# Autodesk Inventor assembly: Short-Cage
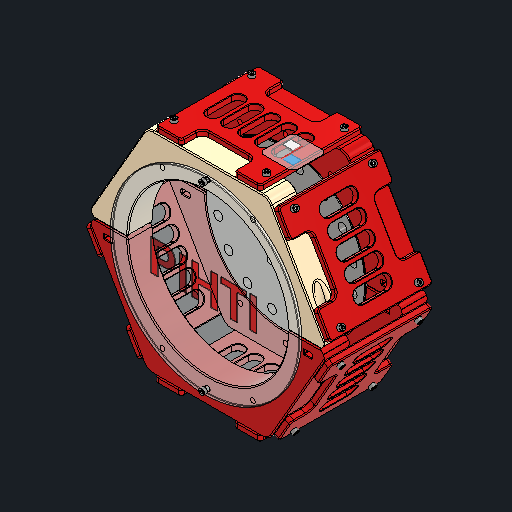
[picture p0: Inventor's stored thumbnail of the model, 512x512]
Saved by Autodesk Inventor 2026 (Build 300175050, 175E)
## iProperties
Created: 2024-07-04
Part Number: Short-Cage
Document SubType Name: Assembly
Designer: kuzmin
Author: kuzmin
## Documents named in this file (8)
- C:\Users\queezz\Dropbox\Drawings\PIHTI\Plasma Vessel\Cathode-Flange-Cage\Short-Cage.iam
- C:\Users\queezz\Dropbox\Drawings\PIHTI\Plasma Vessel\Cathode-Flange-Cage\Baseplate-for-ICF152-flange-outer-part-bottom.ipt
- C:\Users\queezz\Dropbox\Drawings\PIHTI\Plasma Vessel\Cathode-Flange-Cage\Cover-Plate-short-with-bolts.iam
- C:\Users\queezz\Dropbox\Drawings\PIHTI\ContentCenter\CF-parts\CF-Flanges\CF_152-70.ipt
- C:\Users\queezz\Dropbox\Drawings\PIHTI\Plasma Vessel\Cathode-Flange-Cage\cage-disk-lid.ipt
- C:\Users\queezz\Dropbox\Drawings\PIHTI\ContentCenter\Fastners\M3x10-SHCS.ipt
- C:\Users\queezz\Dropbox\Drawings\PIHTI\ContentCenter\Fastners\brass-insert-m3x5.ipt
- C:\Users\queezz\Dropbox\Drawings\PIHTI\Plasma Vessel\Cathode-Flange-Cage\Baseplate-for-ICF152-flange-outer-part-top-v2.ipt
## Components (17 placed, 7 different names)
1. Baseplate-for-ICF152-flange-outer-part-bottom:1 — Rigid:1, Rigid:6, Rigid:7, Rigid:8
2. Baseplate-for-ICF152-flange-outer-part-bottom:2 — Rigid:1, Mate:5, Rigid:3
3. Baseplate-for-ICF152-flange-outer-part-bottom:4 — Mate:5
4. CF_152-70:1 — Rigid:3
5. cage-disk-lid:1 — Rigid:4, Rigid:5, Rigid:9
6. Baseplate-for-ICF152-flange-outer-part-top-v2:1 — Rigid:9
7. JIS B 1176 - Metric M3 x 10:1 — Rigid:5
8. JIS B 1176 - Metric M3 x 10:2 — Rigid:4
9. brass-insert-m3x5:1
10. brass-insert-m3x5:2 — Rigid:6
11. brass-insert-m3x5:3 — Rigid:7
12. brass-insert-m3x5:4
13. Cover-Plate-short-with-bolts:1 [sub-assembly] — Rigid:8
14. Cover-Plate-short-with-bolts:2 [sub-assembly]
15. Cover-Plate-short-with-bolts:3 [sub-assembly]
16. Cover-Plate-short-with-bolts:4 [sub-assembly]
17. Cover-Plate-short-with-bolts:5 [sub-assembly]
## Component patterns: (5 elements, first: Cover-Plate-short-with-bolts:1)
## Relationships (10: WeldJoint 8, Mate 2)
- Rigid:1 [WeldJoint]: Baseplate-for-ICF152-flange-outer-part-bottom:1 ↔ Baseplate-for-ICF152-flange-outer-part-bottom:2
- [Mate]: Baseplate-for-ICF152-flange-outer-part-bottom:1 ↔ Cover-Plate-short-with-bolts:1
- Mate:5: Baseplate-for-ICF152-flange-outer-part-bottom:2 ↔ Baseplate-for-ICF152-flange-outer-part-bottom:4
- Rigid:3 [WeldJoint]: Baseplate-for-ICF152-flange-outer-part-bottom:2 ↔ CF_152-70:1
- Rigid:4 [WeldJoint]: cage-disk-lid:1 ↔ JIS B 1176 - Metric M3 x 10:2
- Rigid:5 [WeldJoint]: cage-disk-lid:1 ↔ JIS B 1176 - Metric M3 x 10:1
- Rigid:6 [WeldJoint]: Baseplate-for-ICF152-flange-outer-part-bottom:1 ↔ brass-insert-m3x5:2
- Rigid:7 [WeldJoint]: Baseplate-for-ICF152-flange-outer-part-bottom:1 ↔ brass-insert-m3x5:3
- Rigid:8 [WeldJoint]: Baseplate-for-ICF152-flange-outer-part-bottom:1 ↔ Cover-Plate-short-with-bolts:1
- Rigid:9 [WeldJoint] (0.5 mm): cage-disk-lid:1 ↔ Baseplate-for-ICF152-flange-outer-part-top-v2:1
